# Autodesk Inventor assembly: 2号螺丝+螺帽
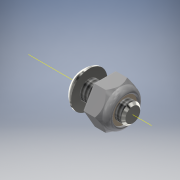
[picture p0: Inventor's stored thumbnail of the model, 180x180]
Saved by Autodesk Inventor 2019.4 (Build 234330000, 330)
## iProperties
Created: 2019-05-20
Part Number: 2号螺丝+螺帽
Material: 常规
Document SubType Name: Assembly
Designer: aresp
Author: aresp
## Documents named in this file (3)
- D:\2019-2020TowerTakeOverCad\ncrCadLib\2号螺丝+螺帽.iam
- C:\TEMP\841588f2-14b1-44e0-8e15-2bb5d77751f4\Screw 8-32 x 0.375'' 二号.ipt
- C:\TEMP\da5afd3b-cf4b-4611-ac24-285cc18734da\防滑螺帽.ipt
## Components (2 placed, 2 different names)
1. Screw 8-32 x 0.375'' 二号:1 — 配合:1, 配合:2
2. 防滑螺帽:1 — 配合:1, 配合:2
## Relationships (2: Mate 2)
- 配合:1 [Mate] (3.15 mm): Screw 8-32 x 0.375'' 二号:1 ↔ 防滑螺帽:1
- 配合:2 [Mate]: Screw 8-32 x 0.375'' 二号:1 ↔ 防滑螺帽:1
